# Autodesk Inventor assembly: WeldedPlenumAssembly
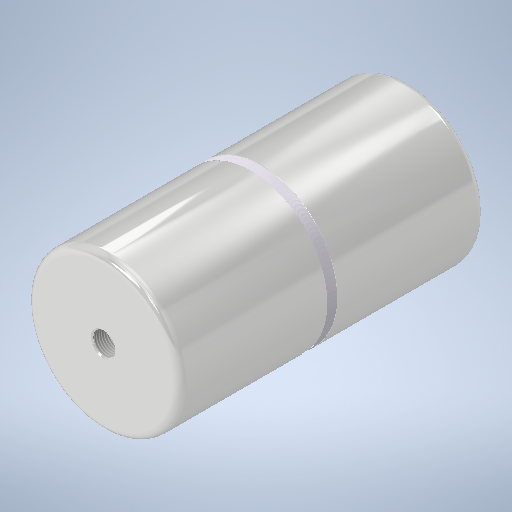
[picture p0: Inventor's stored thumbnail of the model, 512x512]
Saved by Autodesk Inventor 2025.2 (Build 292293000, 293)
## iProperties
Created: 2026-08-04
Part Number: WeldedPlenumAssembly
Document SubType Name: Weldment
Designer: Simon
Weld Material: Welded Aluminum-6061
Author: Simon
## Documents named in this file (3)
- C:\Users\Simon\Projects\MEng Electronics\Development of a Resistojet Thruster\3) Hardware\Resistojet Design\ThrusterV3\Mechanical Drawings\WeldedTankAssembly.iam
- C:\Users\Simon\Projects\MEng Electronics\Development of a Resistojet Thruster\3) Hardware\Resistojet Design\ThrusterV3\Mechanical Drawings\GeneralPressureVesselHalf.ipt
- C:\Users\Simon\Projects\MEng Electronics\Development of a Resistojet Thruster\3) Hardware\Resistojet Design\ThrusterV3\Mechanical Drawings\TankHalf.ipt
## Components (2 placed, 2 different names)
1. GeneralPressureVesselHalf:1 — Mate:1, Mate:2
2. TankHalf:1 — Mate:1, Mate:2
## Relationships (2: Mate 2)
- Mate:1: GeneralPressureVesselHalf:1 ↔ TankHalf:1
- Mate:2: GeneralPressureVesselHalf:1 ↔ TankHalf:1
